# Autodesk Inventor assembly: drive
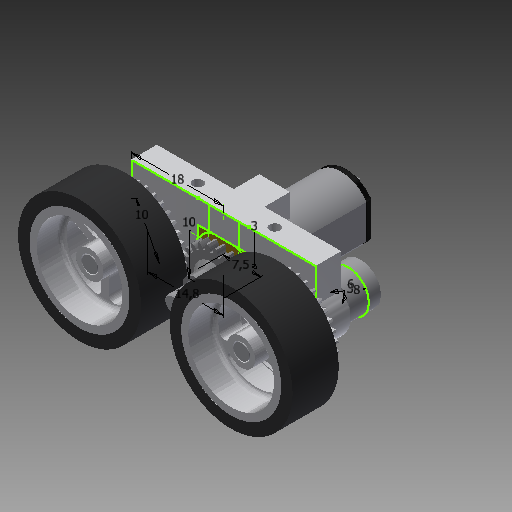
[picture p0: Inventor's stored thumbnail of the model, 512x512]
Saved by Autodesk Inventor 2018 (Build 220112000, 112)
## iProperties
Created: 2018-05-26
Part Number: drive
Material: Ogólny
Document SubType Name: Assembly
Designer: Karol
Author: Karol
## Documents named in this file (10)
- D:\Git\fuckyou\MicromouseDixi\hardware\models\driveRight.iam
- D:\Git\fuckyou\MicromouseDixi\hardware\models\Imported Components\motor_gear\motor_gear.ipt
- D:\Git\fuckyou\MicromouseDixi\hardware\models\Imported Components\wheelv2\wheelv2.ipt
- D:\Git\fuckyou\MicromouseDixi\hardware\models\bearing.ipt
- D:\Git\fuckyou\MicromouseDixi\hardware\models\magnet.ipt
- D:\Git\fuckyou\MicromouseDixi\hardware\models\magnet_holder.ipt
- D:\Git\fuckyou\MicromouseDixi\hardware\models\motor.ipt
- D:\Git\fuckyou\MicromouseDixi\hardware\models\shaft.ipt
- D:\Git\fuckyou\MicromouseDixi\hardware\models\togh.ipt
- D:\Git\fuckyou\MicromouseDixi\hardware\models\tyre.ipt
## Components (15 placed, 9 different names)
1. motor_gear:1 — Sztywne:2
2. bearing:1 — Sztywne:5, Sztywne:16
3. magnet:1 — Sztywne:6
4. magnet_holder:1 — Sztywne:6, Sztywne:16
5. motor:1 — Sztywne:1, Sztywne:2
6. togh:1 — Sztywne:1, Sztywne:15, Sztywne:17
7. shaft:2 — Sztywne:3
8. bearing:2 — Sztywne:5, Obrotowe:3, Sztywne:17
9. wheelv2:2 — Sztywne:3, Sztywne:12, Obrotowe:3
10. bearing:3
11. shaft:3 — Sztywne:9
12. bearing:4 — Obrotowe:2, Sztywne:15
13. wheelv2:3 — Sztywne:9, Sztywne:13, Obrotowe:2
14. tyre:1 — Sztywne:12
15. tyre:2 — Sztywne:13
## Relationships (14: WeldJoint 12, RevoluteJoint 2)
- Sztywne:1 [WeldJoint]: motor:1 ↔ togh:1
- Sztywne:2 [WeldJoint]: motor_gear:1 ↔ motor:1
- Sztywne:3 [WeldJoint]: shaft:2 ↔ wheelv2:2
- Sztywne:5 [WeldJoint]: bearing:1 ↔ bearing:2
- Sztywne:6 [WeldJoint]: magnet:1 ↔ magnet_holder:1
- [WeldJoint]: bearing:3 ↔ bearing:4
- Sztywne:9 [WeldJoint]: shaft:3 ↔ wheelv2:3
- Sztywne:12 [WeldJoint]: wheelv2:2 ↔ tyre:1
- Sztywne:13 [WeldJoint]: wheelv2:3 ↔ tyre:2
- Obrotowe:2 [RevoluteJoint]: bearing:4 ↔ wheelv2:3
- Sztywne:15 [WeldJoint]: togh:1 ↔ bearing:4
- Obrotowe:3 [RevoluteJoint]: bearing:2 ↔ wheelv2:2
- Sztywne:16 [WeldJoint]: bearing:1 ↔ magnet_holder:1
- Sztywne:17 [WeldJoint]: togh:1 ↔ bearing:2
## Named parameters: d9_d6 = 0 mm
